# Autodesk Inventor assembly: Camera assembly
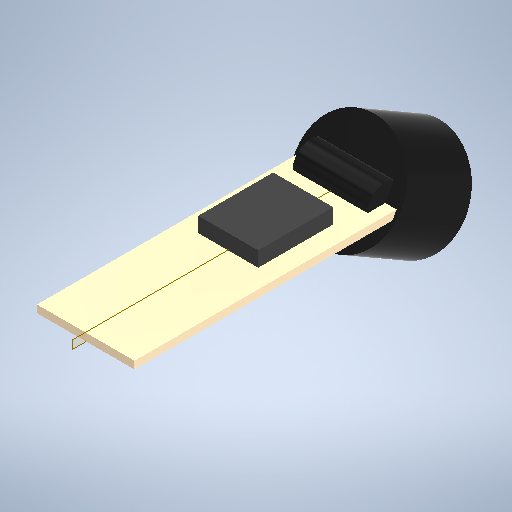
[picture p0: Inventor's stored thumbnail of the model, 512x512]
Saved by Autodesk Inventor 2026.2 (Build 302298010, 298A)
## iProperties
Created: 2026-04-26
Part Number: Camera assembly
Document SubType Name: Assembly
Designer: piete
Author: piete
## Documents named in this file (5)
- C:\Users\piete\Desktop\Skripsie\Documents\Detail Design\Micro Robotics Camera Module\Camera assembly.iam
- C:\Users\piete\Desktop\Skripsie\Documents\Detail Design\Micro Robotics Camera Module\PCB.ipt
- C:\Users\piete\Desktop\Skripsie\Documents\Detail Design\Micro Robotics Camera Module\Epoxy.ipt
- C:\Users\piete\Desktop\Skripsie\Documents\Detail Design\Micro Robotics Camera Module\Electrical Component.ipt
- C:\Users\piete\Desktop\Skripsie\Documents\Detail Design\Micro Robotics Camera Module\Camera and LED sensor.ipt
## Components (4 placed, 4 different names)
1. PCB:1 — Flush:1, Mate:1, Mate:2, Flush:2, Flush:3, Mate:3, Mate:5, Mate:6
2. Epoxy:1 — Flush:1, Mate:1, Mate:2, Mate:4
3. Electrical Component:1 — Flush:2, Flush:3, Mate:3
4. Camera and LED sensor:1 — Mate:4, Mate:5, Mate:6
## Relationships (9: Mate 6, Flush 3)
- Flush:1 (-0.75 mm): PCB:1 ↔ Epoxy:1
- Mate:1: PCB:1 ↔ Epoxy:1
- Mate:2: PCB:1 ↔ Epoxy:1
- Flush:2 (1.25 mm): PCB:1 ↔ Electrical Component:1
- Flush:3 (3 mm): PCB:1 ↔ Electrical Component:1
- Mate:3: PCB:1 ↔ Electrical Component:1
- Mate:4: Epoxy:1 ↔ Camera and LED sensor:1
- Mate:5: PCB:1 ↔ Camera and LED sensor:1
- Mate:6: PCB:1 ↔ Camera and LED sensor:1
